# Autodesk Inventor assembly: uchwyt silnika
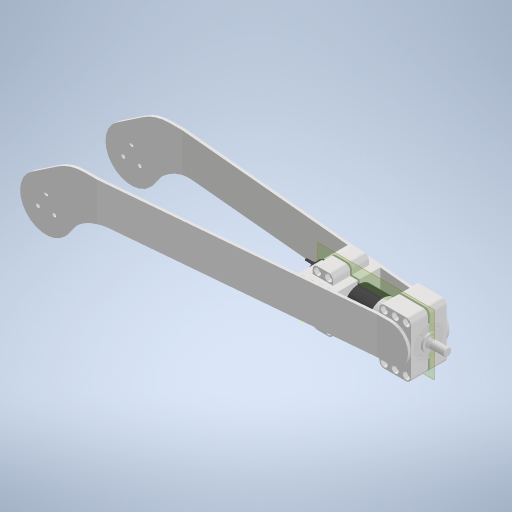
[picture p0: Inventor's stored thumbnail of the model, 512x512]
Saved by Autodesk Inventor 2023 (Build 270158000, 158)
## iProperties
Created: 2023-05-31
Part Number: uchwyt silnika
Document SubType Name: Assembly
Designer: Kamil
Author: Kamil
## iProperties of the stored document MemberDocs/xN3jqom5iJkqy32xoJhld12czHc
Created: 2023-05-31
Part Number: uchwyt silnika
Document SubType Name: Assembly
Designer: Kamil
Author: Kamil
## iProperties of the stored document MemberDocs/xAaaaqucaAaaaaaaaAaaaa5zmVe
Part Number: czlon4_zlozenie — kopia
Document SubType Name: Zespół
Designer: Kamil
Author: Kamil
## Documents named in this file (7)
- C:\Users\Kamil\Desktop\KONARM_2\czlon 4\czlon4_zlozenie — kopia.iam
- C:\Users\Kamil\Desktop\KONARM_2\czlon 4\uchwyt.ipt
- C:\Users\Kamil\Desktop\KONARM_2\czlon 3\Faulhaber 3272G012C R.ipt
- C:\Users\Kamil\Desktop\KONARM_2\czlon 4\uchwyt_MIR.ipt
- C:\Users\Kamil\Desktop\KONARM_2\czlon 4\bok2_MIR.ipt
- C:\Users\Kamil\Desktop\KONARM_2\czlon 4\bok2_MIR_MIR.ipt
- C:\Users\Kamil\Desktop\KONARM_2\czlon 4\czlon4_zlozenie — kopia_SUB.ipt
## Components (5 placed, 5 different names)
1. uchwyt:1 — Równoległe:1, Zestawiające:1, Równoległe:2
2. Faulhaber 3272G012C R:1 — Równoległe:1, Zestawiające:1
3. uchwyt_MIR:1 — Zestawiające:2
4. bok2_MIR:1
5. bok2_MIR_MIR:1
## Relationships (4: Flush 2, Mate 2)
- Równoległe:1 [Flush]: uchwyt:1 ↔ Faulhaber 3272G012C R:1
- Zestawiające:1 [Mate]: uchwyt:1 ↔ Faulhaber 3272G012C R:1
- Równoległe:2 [Flush] (1 mm): uchwyt:1
- Zestawiające:2 [Mate] (1 mm): uchwyt_MIR:1
